# Autodesk Inventor assembly: SPE2V1 Baranda
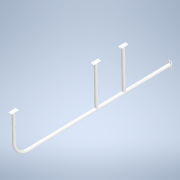
[picture p0: Inventor's stored thumbnail of the model, 180x180]
Saved by Autodesk Inventor 2021 (Build 250183000, 183)
## iProperties
Created: 2026-06-02
Part Number: SPE2V1 Baranda
Document SubType Name: Assembly
Designer: nelso
Author: nelso
## Documents named in this file (4)
- C:\Users\nelso\Desktop\Soporte-Paciente-Espinografia\Workspace\SPE2V1 Baranda.iam
- C:\Users\nelso\Desktop\Soporte-Paciente-Espinografia\Workspace\SP13V1 Tubo Baranda.ipt
- C:\Users\nelso\Desktop\Soporte-Paciente-Espinografia\Workspace\SP12V1 Agarre Baranda.ipt
- C:\Users\nelso\Desktop\Soporte-Paciente-Espinografia\Workspace\SP11V1 Planchuela Baranda.ipt
## Components (7 placed, 3 different names)
1. tubo2-D19.05:1 — Mate:3, Mate:4, Mate:5, Coincidencia:15, Coincidencia:16, Coincidencia:17, Coincidencia:18, Mate:20, Mate:21
2. tubo4-D34.94:1 — Mate:4, Mate:7, Mate:9, Mate:10, Mate:20
3. tubo4-D34.94:2 — Mate:3, Mate:6, Mate:12, Mate:13, Mate:21
4. planchuelaUnion:1 — Mate:8, Mate:9, Mate:10
5. planchuelaUnion:2 — Coincidencia:14, Coincidencia:15, Coincidencia:16
6. planchuelaUnion:3 — Mate:11, Mate:12, Mate:13
7. planchuelaUnion:4 — Coincidencia:17, Coincidencia:18, Coincidencia:19
## Relationships (19: Mate 19)
- Mate:3 (-500 mm): tubo2-D19.05:1 ↔ tubo4-D34.94:2
- Mate:4 (-800 mm): tubo2-D19.05:1 ↔ tubo4-D34.94:1
- Mate:5: tubo2-D19.05:1
- Mate:6: tubo4-D34.94:2
- Mate:7: tubo4-D34.94:1
- Mate:8: planchuelaUnion:1
- Mate:9: tubo4-D34.94:1 ↔ planchuelaUnion:1
- Mate:10: tubo4-D34.94:1 ↔ planchuelaUnion:1
- Mate:11: planchuelaUnion:3
- Mate:12: tubo4-D34.94:2 ↔ planchuelaUnion:3
- Mate:13: tubo4-D34.94:2 ↔ planchuelaUnion:3
- Coincidencia:14 [Mate]: planchuelaUnion:2
- Coincidencia:15 [Mate]: tubo2-D19.05:1 ↔ planchuelaUnion:2
- Coincidencia:16 [Mate]: tubo2-D19.05:1 ↔ planchuelaUnion:2
- Coincidencia:17 [Mate]: tubo2-D19.05:1 ↔ planchuelaUnion:4
- Coincidencia:18 [Mate]: tubo2-D19.05:1 ↔ planchuelaUnion:4
- Coincidencia:19 [Mate]: planchuelaUnion:4
- Mate:20: tubo2-D19.05:1 ↔ tubo4-D34.94:1
- Mate:21: tubo2-D19.05:1 ↔ tubo4-D34.94:2
